# Autodesk Inventor assembly: WE5x4
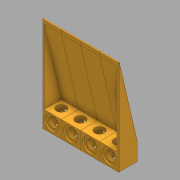
[picture p0: Inventor's stored thumbnail of the model, 180x180]
Saved by Autodesk Inventor 2019.3 (Build 233278000, 278)
## iProperties
Created: 2019-02-07
Part Number: WE5x4
Document SubType Name: Assembly
Designer: Varga Daniel
Wedge_assembly_length: 50,000 mm
Author: Varga Daniel
## Documents named in this file (6)
- C:\!_Dani\!_cloud\OneDrive\!_munka\Revolution\RevvyDemoKit\Structural parts\Wedges\WE2+x1+\WE5x4.iam
- C:\!_Dani\!_cloud\OneDrive\!_munka\Revolution\RevvyDemoKit\Structural parts\Wedges\Wedge_base.ipt
- C:\!_Dani\!_cloud\OneDrive\!_munka\Revolution\RevvyDemoKit\Structural parts\Wedges\Wedge_base\Wedge_base-right.ipt
- C:\!_Dani\!_cloud\OneDrive\!_munka\Revolution\RevvyDemoKit\Structural parts\Wedges\Wedge_base\Wedge_base-inner.ipt
- C:\!_Dani\!_cloud\OneDrive\!_munka\Revolution\RevvyDemoKit\Structural parts\Wedges\Wedge_base\Wedge_base-left.ipt
- C:\!_Dani\!_cloud\OneDrive\!_munka\Revolution\RevvyDemoKit\Structural parts\Wedges\WE2+x1+.iam
## Components (4 placed, 3 different names)
1. Wedge_base-left:1 — Flush:1, Flush:2, Flush:3, Flush:4, Mate:1, Mate:2
2. Wedge_base-right:2 — Flush:2, Flush:4, Mate:1
3. Wedge_base-inner:3 — Flush:1, Flush:3, Mate:2
4. Wedge_base-inner:6
## Component patterns: (2 elements, first: Wedge_base-inner:3)
## Relationships (6: Flush 4, Mate 2)
- Flush:1: Wedge_base-left:1 ↔ Wedge_base-inner:3
- Flush:2: Wedge_base-left:1 ↔ Wedge_base-right:2
- Flush:3: Wedge_base-left:1 ↔ Wedge_base-inner:3
- Flush:4: Wedge_base-left:1 ↔ Wedge_base-right:2
- Mate:1 (20 mm): Wedge_base-left:1 ↔ Wedge_base-right:2
- Mate:2: Wedge_base-left:1 ↔ Wedge_base-inner:3
